(part 1 of 2)
# Autodesk Inventor assembly: ATLAS ASSEMBLY
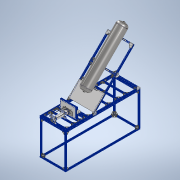
[picture p0: Inventor's stored thumbnail of the model, 180x180]
Saved by Autodesk Inventor 2021 (Build 250183000, 183)
## iProperties
Created: 2021-09-10
Part Number: ATLAS ASSEMBLY
Document SubType Name: Assembly
Designer: Alex Clay
Author: Alex Clay
## Documents named in this file (38)
- C:\Users\alexc\Embry-Riddle Aeronautical University\Kingsberry, Kyle A. - Odyssey\ATLAS V1\ATLAS ASSEMBLY.iam
- C:\Users\alexc\Embry-Riddle Aeronautical University\Kingsberry, Kyle A. - Odyssey\ATLAS V1\4040 6ft.ipt
- C:\Users\alexc\Embry-Riddle Aeronautical University\Kingsberry, Kyle A. - Odyssey\ATLAS V1\4040 3.5ft.ipt
- C:\Users\alexc\Embry-Riddle Aeronautical University\Kingsberry, Kyle A. - Odyssey\ATLAS V1\4040 2.5ft.ipt
- C:\Users\alexc\Embry-Riddle Aeronautical University\Kingsberry, Kyle A. - Odyssey\ATLAS V1\4080 6ft.ipt
- C:\Users\alexc\Embry-Riddle Aeronautical University\Kingsberry, Kyle A. - Odyssey\ATLAS V1\4 Hole Bracket.ipt
- C:\Users\alexc\Embry-Riddle Aeronautical University\Kingsberry, Kyle A. - Odyssey\ATLAS V1\4040 1ft.ipt
- C:\Users\alexc\Embry-Riddle Aeronautical University\Kingsberry, Kyle A. - Odyssey\ATLAS V1\4040 1.5ft.ipt
- C:\Users\alexc\Embry-Riddle Aeronautical University\Kingsberry, Kyle A. - Odyssey\ATLAS V1\45 Plate.ipt
- C:\Users\alexc\Embry-Riddle Aeronautical University\Kingsberry, Kyle A. - Odyssey\ATLAS V1\4040 angled.ipt
- C:\Users\alexc\Embry-Riddle Aeronautical University\Kingsberry, Kyle A. - Odyssey\ATLAS V1\4080 2.5ft.ipt
- C:\Users\alexc\Embry-Riddle Aeronautical University\Kingsberry, Kyle A. - Odyssey\ATLAS V1\90 Plate.ipt
- C:\Users\alexc\Embry-Riddle Aeronautical University\Kingsberry, Kyle A. - Odyssey\ATLAS V1\ODSY-0007-003.ipt
- C:\Users\alexc\Embry-Riddle Aeronautical University\Kingsberry, Kyle A. - Odyssey\ATLAS V1\Odyssey Bushing.ipt
- C:\Users\alexc\Embry-Riddle Aeronautical University\Kingsberry, Kyle A. - Odyssey\ATLAS V1\ODSY-0007-001.ipt
- C:\Users\alexc\Embry-Riddle Aeronautical University\Kingsberry, Kyle A. - Odyssey\ATLAS V1\8080 2.5ft.ipt
- C:\Users\alexc\Embry-Riddle Aeronautical University\Kingsberry, Kyle A. - Odyssey\ATLAS V1\ODSY-0007-002.ipt
- C:\Users\alexc\Embry-Riddle Aeronautical University\Kingsberry, Kyle A. - Odyssey\ATLAS V1\ODSY-0003 (COMBUSTION CHAMBER)\ODSY-0003.iam
- C:\Users\alexc\Embry-Riddle Aeronautical University\Kingsberry, Kyle A. - Odyssey\ATLAS V1\Load Cell.ipt
- C:\Users\alexc\Embry-Riddle Aeronautical University\Kingsberry, Kyle A. - Odyssey\ATLAS V1\ODSY-0007-004.ipt
- C:\Users\alexc\Embry-Riddle Aeronautical University\Kingsberry, Kyle A. - Odyssey\ATLAS V1\95412A566 Short Threaded Rod.ipt
- C:\Users\alexc\Embry-Riddle Aeronautical University\Kingsberry, Kyle A. - Odyssey\ATLAS V1\98804A029 Long Threaded Rod.ipt
- C:\Users\alexc\Embry-Riddle Aeronautical University\Kingsberry, Kyle A. - Odyssey\ATLAS V1\92196A801 Load Cell Bolt.ipt
- C:\Users\alexc\Embry-Riddle Aeronautical University\Kingsberry, Kyle A. - Odyssey\ATLAS V1\92141A029 0.25 Washer.ipt
- C:\Users\alexc\Embry-Riddle Aeronautical University\Kingsberry, Kyle A. - Odyssey\ATLAS V1\91292A209 Bottom Holder Screw.ipt
- C:\Users\alexc\Embry-Riddle Aeronautical University\Kingsberry, Kyle A. - Odyssey\ATLAS V1\98689A116 Bottom Holder Washer.ipt
- C:\Users\alexc\Embry-Riddle Aeronautical University\Kingsberry, Kyle A. - Odyssey\ATLAS V1\91845A029 0.25 Nut.ipt
- C:\Users\alexc\Embry-Riddle Aeronautical University\Kingsberry, Kyle A. - Odyssey\ATLAS V1\92510A475 Spacer.ipt
- C:\Users\alexc\Embry-Riddle Aeronautical University\Kingsberry, Kyle A. - Odyssey\ATLAS V1\92196A551 Engine Bolts.ipt
- C:\Users\alexc\Embry-Riddle Aeronautical University\Kingsberry, Kyle A. - Odyssey\ATLAS V1\90945A760 Washers For Engine.ipt
- C:\Users\alexc\Embry-Riddle Aeronautical University\Kingsberry, Kyle A. - Odyssey\ATLAS V1\91831A029 Lock Nuts For Engine.ipt
- C:\Users\alexc\Embry-Riddle Aeronautical University\Kingsberry, Kyle A. - Odyssey\ATLAS V1\Tank Uprights.ipt
- C:\Users\alexc\Embry-Riddle Aeronautical University\Kingsberry, Kyle A. - Odyssey\ATLAS V1\Tank Holder.ipt
- C:\Users\alexc\Embry-Riddle Aeronautical University\Kingsberry, Kyle A. - Odyssey\ATLAS V1\Tank Upright Support.ipt
- C:\Users\alexc\Embry-Riddle Aeronautical University\Kingsberry, Kyle A. - Odyssey\ATLAS V1\45 splicer.ipt
- C:\Users\alexc\Embry-Riddle Aeronautical University\Kingsberry, Kyle A. - Odyssey\ATLAS V1\40-4340.ipt
- C:\Users\alexc\Embry-Riddle Aeronautical University\Kingsberry, Kyle A. - Odyssey\ATLAS V1\Odyssey Fluids Panel.ipt
- C:\Users\alexc\Embry-Riddle Aeronautical University\Kingsberry, Kyle A. - Odyssey\ATLAS V1\ODSY-0004 (TANK)\Weld Assembly.iam
## Components (292 placed, 37 different names)
1. 4040 6ft:1 — Flush:3, Flush:4, Flush:7, Flush:8, Mate:3, Flush:11, Flush:12, Mate:5, Mate:10, Mate:28, Mate:31, Flush:39, Mate:33, Mate:36, Flush:42
2. 4040 6ft:2 — Flush:1, Mate:1, Flush:2, Flush:3, Flush:4, Flush:5, Flush:6, Mate:2, Flush:9, Flush:10, Mate:4, Mate:6, Flush:13, Flush:14, Mate:9, Flush:19, Flush:20, Mate:20, Mate:25, Mate:39, Flush:43, Mate:42
3. 4040 3.5ft:1 — Flush:7, Flush:8, Mate:3, Mate:12, Flush:23, Flush:24, Mate:27, Flush:37, Mate:29, Flush:38, Flush:49, Mate:52, Flush:93
4. 4040 3.5ft:2 — Flush:5, Flush:6, Mate:2, Flush:21, Flush:22, Mate:11, Mate:21, Flush:34, Mate:22, Flush:35, Mate:44, Flush:46, Flush:92, Flush:94
5. 4040 3.5ft:3 — Flush:9, Flush:10, Mate:4, Mate:38, Mate:40, Mate:56, Mate:59, Flush:99
6. 4040 3.5ft:4 — Flush:11, Flush:12, Mate:5, Mate:32, Flush:40, Mate:34, Mate:65, Mate:67, Flush:57, Flush:95, Flush:96
7. 4040 2.5ft:1 — Mate:6, Flush:13, Flush:14, Mate:35, Flush:41, Mate:37, Mate:41, Flush:44, Mate:43, Flush:45
8. 4040 2.5ft:2 — Mate:9, Flush:19, Flush:20, Mate:10, Mate:23, Mate:24, Flush:36, Mate:26, Mate:30
9. 4080 6ft:1 — Flush:21, Flush:22, Mate:11, Mate:15, Flush:29, Mate:17, Flush:31, Mate:45, Mate:46, Mate:48, Flush:48, Flush:52, Mate:58, Flush:53, Mate:60, Mate:70, Mate:71, Mate:82, Mate:83, Mate:84, Mate:85, Mate:86, Mate:87, Flush:98, Flush:100, Flush:101, Mate:204, Flush:102, Flush:103, Mate:207, Flush:104, Flush:105, Flush:108, Flush:109, Mate:212, Flush:112, Mate:217, Flush:113, Mate:241, Mate:242, Flush:122, Flush:123, Mate:257, Mate:259, Mate:261, Mate:263, Mate:492, Mate:518, Mate:545, Mate:584, Mate:585, Mate:586
10. 4080 6ft:2 — Mate:12, Flush:23, Flush:24, Mate:50, Mate:53, Flush:50, Mate:55, Mate:62, Mate:66, Mate:98, Mate:99, Mate:102, Mate:103, Mate:104, Mate:105, Mate:106, Mate:107, Flush:91, Flush:97, Flush:106, Flush:107, Flush:110, Flush:111, Mate:245, Mate:247, Mate:249, Mate:251, Mate:493, Mate:494, Mate:495, Mate:520, Mate:544, Mate:583, Mate:588, Mate:589, Flush:187
11. 4040 2.5ft:5 — Mate:15, Flush:29, Mate:68, Mate:69, Flush:58, Flush:59, Mate:88, Mate:89, Flush:76, Flush:77, Mate:184, Mate:185, Mate:289
12. 4040 2.5ft:6 — Mate:17, Flush:31, Mate:76, Mate:77, Flush:62, Flush:63, Mate:94, Mate:95, Flush:68, Flush:69
13. 4 Hole Bracket:1 — Mate:24, Mate:25, Flush:36
14. 4 Hole Bracket:2 — Mate:22, Mate:23, Flush:35
15. 4 Hole Bracket:3 — Mate:20, Mate:21, Flush:34
16. 4 Hole Bracket:4 — Mate:44, Mate:45, Flush:46
17. 4 Hole Bracket:5 — Mate:48, Flush:48, Mate:205
18. 4 Hole Bracket:6 — Mate:46, Flush:92, Flush:94
19. 4 Hole Bracket:7 — Mate:30, Mate:31, Flush:39
20. 4 Hole Bracket:8 — Mate:28, Mate:29, Flush:38
21. 4 Hole Bracket:9 — Mate:26, Mate:27, Flush:37
22. 4 Hole Bracket:10 — Mate:34, Mate:35, Flush:41
23. 4 Hole Bracket:11 — Mate:38, Mate:39, Flush:43
24. 4 Hole Bracket:12 — Mate:32, Mate:33, Flush:40
25. 4 Hole Bracket:13 — Mate:36, Mate:37, Flush:42
26. 4 Hole Bracket:14 — Mate:40, Mate:41, Flush:44
27. 4 Hole Bracket:15 — Mate:42, Mate:43, Flush:45
28. 4 Hole Bracket:16 — Mate:62, Flush:97, Mate:209
29. 4 Hole Bracket:17 — Mate:65, Flush:95, Flush:96
30. 4 Hole Bracket:18 — Mate:66, Mate:67, Flush:57
31. 4 Hole Bracket:19 — Mate:60, Flush:98, Mate:208
32. 4 Hole Bracket:20 — Mate:58, Mate:59, Flush:53
33. 4 Hole Bracket:21 — Mate:56, Flush:52, Flush:99
34. 4 Hole Bracket:22 — Mate:50, Flush:49, Flush:93
35. 4 Hole Bracket:23 — Mate:55, Flush:91, Mate:206
36. 4 Hole Bracket:24 — Mate:52, Mate:53, Flush:50
37. 4 Hole Bracket:25 — Mate:88, Mate:107, Flush:76
38. 4 Hole Bracket:26 — Mate:89, Mate:106, Flush:77
39. 4 Hole Bracket:27 — Mate:105, Flush:111, Mate:220
40. 4 Hole Bracket:28 — Mate:104, Flush:110, Mate:221
41. 4 Hole Bracket:29 — Mate:103, Flush:107, Mate:215
42. 4 Hole Bracket:30 — Mate:102, Flush:106, Mate:216
43. 4 Hole Bracket:31 — Mate:94, Mate:99, Flush:69
44. 4 Hole Bracket:32 — Mate:95, Mate:98, Flush:68
45. 4 Hole Bracket:37 — Mate:77, Mate:83, Flush:63
46. 4 Hole Bracket:38 — Mate:76, Mate:82, Flush:62
47. 4 Hole Bracket:39 — Mate:85, Flush:105, Mate:214
48. 4 Hole Bracket:40 — Mate:84, Flush:104, Mate:213
49. 4 Hole Bracket:41 — Mate:87, Flush:109, Mate:219
50. 4 Hole Bracket:42 — Mate:86, Flush:108, Mate:218
51. 4 Hole Bracket:43 — Mate:69, Mate:71, Flush:58
52. 4 Hole Bracket:44 — Mate:68, Mate:70, Flush:59
53. 4040 1ft:1 — Mate:110, Flush:80, Flush:81, Mate:133, Flush:85, Mate:167, Mate:176, Mate:177, Mate:178, Mate:210, Mate:229
54. 4040 1ft:2 — Mate:111, Flush:82, Flush:83, Mate:112, Mate:113, Mate:129, Mate:173, Mate:211, Mate:227, Flush:116, Mate:228, Flush:119, Mate:232
55. 4040 1.5ft:1 — Mate:110, Flush:80, Flush:81, Mate:111, Flush:82, Flush:83, Mate:186, Mate:187, Flush:117, Flush:118
56. 45 Plate:2 — Mate:112, Mate:113, Mate:126, Mate:127, Mate:128
57. 4040 angled:1 — Mate:126, Mate:127, Mate:128, Mate:129, Mate:226, Mate:343
58. 4040 angled:2 — Mate:133, Flush:85, Mate:179, Mate:533
59. 90 Plate:2 — Mate:167, Mate:210, Mate:229, Mate:230
60. 90 Plate:4 — Mate:173, Mate:211, Mate:228, Mate:231
61. 45 Plate:3 — Mate:176, Mate:177, Mate:178, Mate:179
62. ODSY-0007-003:1 — Mate:186, Mate:233, Mate:282, Mate:283, Mate:284, Mate:285, Mate:286, Mate:287, Mate:288, Angle:1, Mate:293, Mate:294, Mate:307, Mate:308, Mate:312, Mate:313, Mate:377, Mate:378, Mate:384, Mate:387, Mate:456
63. ODSY-0007-003:2 — Mate:184, Mate:185, Mate:187, Mate:195, Mate:196, Mate:197, Mate:279, Mate:280, Mate:281, Mate:289, Mate:291, Mate:292, Mate:309, Mate:310, Mate:311, Mate:314, Mate:376, Mate:379, Mate:385, Mate:386, Mate:456
64. Odyssey Bushing:1 — Mate:195, Mate:196, Mate:197
65. 8080 2.5ft:1 — Flush:100, Flush:101, Mate:204, Mate:205, Mate:206, Mate:233, Mate:288
66. 8080 2.5ft:2 — Flush:102, Flush:103, Mate:207, Mate:208, Mate:209
67. 8080 2.5ft:3 — Mate:217, Flush:113, Mate:218, Mate:219, Mate:220, Mate:221, Mate:226, Mate:343, Mate:533
68. 4080 2.5ft:1 — Mate:212, Flush:112, Mate:213, Mate:214, Mate:215, Mate:216, Mate:227, Flush:116, Mate:230, Mate:231, Flush:117
69. ODSY-0007-001:1 — Flush:118, Flush:119, Mate:232, Mate:275, Mate:276, Mate:331, Mate:332, Mate:334, Mate:337, Mate:368, Mate:369, Mate:370, Mate:371, Mate:466, Mate:472
70. ODSY-0007-002:1 — Mate:268, Mate:269, Mate:342, Mate:467, Mate:468, Mate:469, Mate:470, Mate:481, Mate:484, Mate:486
71. 4040 2.5ft:8 — Mate:241, Flush:123, Mate:244, Flush:124, Mate:246, Flush:125, Mate:256, Flush:130, Mate:258, Flush:131
72. 4040 2.5ft:9 — Mate:242, Flush:122, Mate:248, Flush:126, Mate:250, Flush:127, Mate:260, Flush:132, Mate:262, Flush:133
73. 4 Hole Bracket:45 — Mate:244, Flush:124, Mate:245
74. 4 Hole Bracket:46 — Mate:246, Flush:125, Mate:247
75. 4 Hole Bracket:48 — Mate:248, Flush:126, Mate:249
76. 4 Hole Bracket:49 — Mate:250, Flush:127, Mate:251
77. 4 Hole Bracket:51 — Mate:258, Flush:131, Mate:259
78. 4 Hole Bracket:52 — Mate:256, Flush:130, Mate:257
79. 4 Hole Bracket:55 — Mate:262, Flush:133, Mate:263
80. 4 Hole Bracket:56 — Mate:260, Flush:132, Mate:261
81. Combustion Chamber Assembly:1 [sub-assembly] — Mate:268, Mate:269, Mate:488, Mate:489
82. Load Cell:1 — Mate:275, Mate:276, Mate:469
83. Odyssey Bushing:2 — Mate:279, Mate:280, Mate:281
84. Odyssey Bushing:3 — Mate:285, Mate:286, Mate:287
85. Odyssey Bushing:4 — Mate:282, Mate:283, Mate:284
86. ODSY-0007-004:1 — Angle:1, Mate:293, Mate:294, Mate:295, Mate:296, Mate:297, Mate:298, Mate:299, Mate:300, Mate:350, Mate:351, Mate:357, Mate:359, Mate:374, Mate:375, Mate:471, Mate:476, Mate:478
87. ODSY-0007-004:2 — Mate:291, Mate:292, Mate:301, Mate:302, Mate:303, Mate:304, Mate:305, Mate:306, Mate:319, Mate:320, Mate:345, Mate:347, Mate:353, Mate:355, Mate:372, Mate:373, Mate:474, Mate:480
88. Odyssey Bushing:5 — Mate:298, Mate:299, Mate:300
89. Odyssey Bushing:6 — Mate:295, Mate:296, Mate:297
90. Odyssey Bushing:7 — Mate:304, Mate:305, Mate:306
91. Odyssey Bushing:8 — Mate:301, Mate:302, Mate:303
92. 95412A566 Short Threaded Rod:1 — Mate:310, Mate:311, Mate:344, Mate:400, Mate:401, Mate:473
93. 95412A566 Short Threaded Rod:2 — Mate:307, Mate:312, Mate:348, Mate:392, Mate:393, Mate:475
94. 95412A566 Short Threaded Rod:3 — Mate:309, Mate:314, Mate:346, Mate:404, Mate:405, Mate:479
95. 95412A566 Short Threaded Rod:4 — Mate:308, Mate:313, Mate:349, Mate:397, Mate:398, Mate:477
96. 98804A029 Long Threaded Rod:1 — Mate:319, Mate:352, Mate:354, Mate:356, Mate:358, Mate:366, Mate:367, Mate:408, Mate:409, Mate:414, Mate:415, Mate:424, Mate:425, Mate:426, Mate:427, Mate:444, Mate:445, Mate:446, Mate:447, Flush:150, Flush:151, Flush:152, Mate:471, Mate:472
97. 98804A029 Long Threaded Rod:2 — Mate:320, Mate:360, Mate:361, Mate:362, Mate:363, Mate:364, Mate:365, Mate:410, Mate:411, Mate:412, Mate:413, Mate:428, Mate:429, Mate:430, Mate:431, Mate:440, Mate:441, Mate:442, Mate:443, Flush:150
98. 92196A801 Load Cell Bolt:1 — Mate:331, Mate:333, Mate:335, Mate:341, Mate:457, Mate:458, Mate:465, Mate:467
99. 92196A801 Load Cell Bolt:2 — Mate:332, Mate:336, Mate:338, Mate:339, Mate:461, Mate:463, Mate:468
100. 92141A029 0.25 Washer:1 — Mate:333, Mate:334, Mate:335
101. 92141A029 0.25 Washer:2 — Mate:336, Mate:337, Mate:338
102. 92141A029 0.25 Washer:3 — Mate:341, Mate:342, Mate:459
103. 92141A029 0.25 Washer:4 — Mate:339, Mate:462, Mate:470
104. 92141A029 0.25 Washer:5 — Mate:346, Mate:347, Mate:407
105. 92141A029 0.25 Washer:6 — Mate:348, Mate:351, Mate:394
106. 92141A029 0.25 Washer:7 — Mate:344, Mate:345, Mate:403
107. 92141A029 0.25 Washer:8 — Mate:349, Mate:350, Mate:396
108. 92141A029 0.25 Washer:9 — Mate:356, Mate:357, Mate:418
109. 92141A029 0.25 Washer:10 — Mate:358, Mate:359, Mate:416
110. 92141A029 0.25 Washer:11 — Mate:354, Mate:355, Mate:434
111. 92141A029 0.25 Washer:12 — Mate:352, Mate:353, Mate:432
112. 92141A029 0.25 Washer:13 — Mate:360, Mate:374, Mate:420
113. 92141A029 0.25 Washer:14 — Mate:361, Mate:375, Mate:422
114. 92141A029 0.25 Washer:15 — Mate:362, Mate:372, Mate:436
115. 92141A029 0.25 Washer:16 — Mate:363, Mate:373, Mate:438
116. 92141A029 0.25 Washer:17 — Mate:364, Mate:368, Mate:455
117. 92141A029 0.25 Washer:18 — Mate:365, Mate:371, Mate:451
118. 92141A029 0.25 Washer:19 — Mate:367, Mate:369, Mate:452
119. 92141A029 0.25 Washer:20 — Mate:366, Mate:370, Mate:449
120. 91292A209 Bottom Holder Screw:1 — Mate:377, Mate:381, Mate:388
121. 91292A209 Bottom Holder Screw:2 — Mate:376, Mate:380, Mate:389
122. 91292A209 Bottom Holder Screw:3 — Mate:379, Mate:383, Mate:391
123. 91292A209 Bottom Holder Screw:4 — Mate:378, Mate:382, Mate:390
124. 98689A116 Bottom Holder Washer:1 — Mate:381, Mate:387, Mate:388
125. 98689A116 Bottom Holder Washer:2 — Mate:380, Mate:386, Mate:389
126. 98689A116 Bottom Holder Washer:3 — Mate:382, Mate:384, Mate:390
127. 98689A116 Bottom Holder Washer:4 — Mate:383, Mate:385, Mate:391
128. 91845A029 0.25 Nut:1 — Mate:404, Mate:406
129. 91845A029 0.25 Nut:2 — Mate:393, Flush:136, Mate:395
130. 91845A029 0.25 Nut:3 — Mate:400, Flush:138, Mate:402, Mate:403
131. 91845A029 0.25 Nut:4 — Mate:392, Flush:136, Mate:394, Mate:395
132. 91845A029 0.25 Nut:5 — Mate:398, Flush:137, Mate:399
133. 91845A029 0.25 Nut:6 — Mate:405, Mate:406, Mate:407
134. 91845A029 0.25 Nut:7 — Mate:401, Flush:138, Mate:402
135. 91845A029 0.25 Nut:8 — Mate:396, Mate:397, Flush:137, Mate:399
136. 91845A029 0.25 Nut:9 — Mate:415, Flush:139, Mate:416, Mate:417
137. 91845A029 0.25 Nut:10 — Mate:414, Flush:139, Mate:417
138. 91845A029 0.25 Nut:11 — Mate:413, Mate:421, Flush:141
139. 91845A029 0.25 Nut:12 — Mate:412, Mate:420, Mate:421, Flush:141
140. 91845A029 0.25 Nut:13 — Mate:410, Mate:422, Mate:423, Flush:142
141. 91845A029 0.25 Nut:14 — Mate:411, Mate:423, Flush:142
142. 91845A029 0.25 Nut:15 — Mate:408, Mate:418, Mate:419, Flush:140
143. 91845A029 0.25 Nut:16 — Mate:409, Mate:419, Flush:140, Flush:151
144. 91845A029 0.25 Nut:17 — Mate:424, Flush:146, Mate:432, Mate:433
145. 91845A029 0.25 Nut:18 — Mate:425, Flush:146, Mate:433
146. 91845A029 0.25 Nut:19 — Mate:426, Flush:145, Mate:434, Mate:435
147. 91845A029 0.25 Nut:20 — Mate:427, Flush:145, Mate:435
148. 91845A029 0.25 Nut:21 — Mate:429, Flush:144, Mate:437
149. 91845A029 0.25 Nut:22 — Mate:428, Flush:144, Mate:436, Mate:437
150. 91845A029 0.25 Nut:23 — Mate:431, Flush:143, Mate:438, Mate:439
151. 91845A029 0.25 Nut:24 — Mate:430, Flush:143, Mate:439
152. 91845A029 0.25 Nut:25 — Mate:445, Mate:453
153. 91845A029 0.25 Nut:26 — Mate:444, Mate:452, Mate:453
154. 91845A029 0.25 Nut:27 — Mate:447, Flush:147, Mate:448, Mate:449
155. 91845A029 0.25 Nut:28 — Mate:446, Flush:147, Mate:448, Flush:152
156. 91845A029 0.25 Nut:29 — Mate:440, Mate:450, Flush:148, Mate:451
157. 91845A029 0.25 Nut:30 — Mate:441, Mate:450, Flush:148
158. 91845A029 0.25 Nut:31 — Mate:442, Mate:454, Flush:149, Mate:455
159. 91845A029 0.25 Nut:32 — Mate:443, Mate:454, Flush:149
160. 91845A029 0.25 Nut:33 — Mate:461, Mate:462, Flush:154, Mate:464
161. 91845A029 0.25 Nut:34 — Mate:463, Flush:154, Mate:464
162. 91845A029 0.25 Nut:35 — Mate:457, Flush:153, Mate:459, Mate:460
163. 91845A029 0.25 Nut:36 — Mate:458, Flush:153, Mate:460
164. Load Cell:2 — Mate:465, Mate:466
165. 92510A475 Spacer:1 — Mate:475, Mate:476
166. 92510A475 Spacer:2 — Mate:473, Mate:474
167. 92510A475 Spacer:3 — Mate:479, Mate:480
168. 92510A475 Spacer:4 — Mate:477, Mate:478
169. 45 Plate:4 — Mate:493, Flush:155, Flush:156, Mate:494, Mate:495, Mate:496, Mate:498, Mate:499
170. 45 Plate:5 — Mate:492, Flush:155, Flush:156, Mate:497, Mate:501, Mate:502, Mate:503
171. Tank Uprights:1 — Mate:496, Mate:498, Mate:499, Mate:506, Flush:159, Flush:161, Flush:163, Mate:515, Mate:536, Mate:537, Mate:542, Flush:169, Flush:170, Mate:552, Flush:176, Mate:556, Mate:561, Flush:180, Mate:563, Flush:181, Mate:567, Flush:183, Mate:570, Mate:571, Mate:572, Mate:573, Mate:578, Flush:185
172. Tank Uprights:2 — Mate:497, Mate:501, Mate:502, Mate:503, Mate:507, Flush:160, Flush:164, Mate:516, Mate:528, Mate:539, Mate:540, Mate:543, Flush:171, Flush:172, Mate:546, Flush:173, Mate:551, Mate:554, Flush:177, Mate:559, Flush:179, Mate:565, Flush:182, Mate:569, Flush:184, Mate:577
173. 4040 2.5ft:12 — Mate:507, Flush:160, Mate:508, Mate:512, Flush:161, Mate:532, Mate:550, Flush:175, Mate:553, Mate:574, Mate:575, Mate:576
174. 4040 2.5ft:13 — Mate:506, Flush:159, Mate:509, Mate:513, Mate:532, Mate:555, Mate:557, Flush:178, Mate:558, Mate:560
175. Tank Holder:1 — Mate:509, Mate:513, Mate:528, Mate:580, Mate:581
176. Tank Holder:2 — Mate:508, Mate:512, Mate:580, Mate:582
177. Tank Upright Support:1 — Flush:164, Mate:516, Mate:517, Flush:165, Flush:166, Mate:535, Mate:541, Mate:587
178. Tank Upright Support:2 — Flush:163, Mate:515, Mate:519, Flush:167, Flush:168, Mate:534, Mate:538, Mate:590
179. 45 splicer:1 — Mate:517, Flush:165, Flush:166, Mate:518
180. 45 splicer:2 — Mate:519, Flush:167, Flush:168, Mate:520
181. 40-4340:1 — Mate:534, Mate:536, Mate:537, Mate:538
182. 40-4340:2 — Mate:535, Mate:539, Mate:540, Mate:541
183. 45 splicer:3 — Mate:543, Flush:171, Flush:172, Mate:545
184. 45 splicer:4 — Mate:542, Flush:169, Flush:170, Mate:544, Mate:579
185. 4040 2.5ft:14 — Mate:546, Flush:173, Mate:548, Flush:174, Mate:562, Mate:564, Mate:566, Mate:568, Flush:186
186. Tank Holder:3 — Mate:548, Flush:174, Mate:581
187. 4 Hole Bracket:57 — Mate:550, Mate:551, Flush:175
188. 4 Hole Bracket:58 — Mate:552, Mate:553, Flush:176
189. 4 Hole Bracket:59 — Mate:554, Mate:555, Flush:177
190. 4 Hole Bracket:60 — Mate:568, Mate:569, Flush:184
191. 4 Hole Bracket:61 — Mate:556, Mate:557, Flush:178
192. 4 Hole Bracket:62 — Mate:560, Mate:561, Flush:180
193. 4 Hole Bracket:63 — Mate:558, Mate:559, Flush:179
194. 4 Hole Bracket:64 — Mate:562, Mate:563, Flush:181
195. 4 Hole Bracket:65 — Mate:564, Mate:565, Flush:182
196. 4 Hole Bracket:66 — Mate:566, Mate:567, Flush:183
197. 45 Plate:6 — Mate:570, Mate:571, Mate:572, Mate:573
198. 45 Plate:7 — Mate:574, Mate:575, Mate:576, Mate:577
199. Odyssey Fluids Panel:1 — Mate:578, Mate:579, Flush:185, Flush:186
200. Weld Assembly:1 [sub-assembly] — Mate:582
201. 45 Plate:8 — Mate:584, Mate:585, Mate:586, Mate:587
202. 45 Plate:9 — Mate:583, Mate:588, Mate:589, Mate:590, Flush:187
203. 92196A551 Engine Bolts:1 — Mate:481, Mate:482, Mate:483, Mate:485, Mate:487, Mate:490
204. 90945A760 Washers For Engine:1 — Mate:482, Mate:483, Mate:484
205. 90945A760 Washers For Engine:2 — Mate:485, Mate:486, Mate:488
206. 90945A760 Washers For Engine:3 — Mate:487, Mate:489, Mate:491
207. 91831A029 Lock Nuts For Engine:1 — Mate:490, Mate:491
208. 92196A551 Engine Bolts:2
209. 90945A760 Washers For Engine:4
210. 90945A760 Washers For Engine:5
211. 90945A760 Washers For Engine:6
212. 91831A029 Lock Nuts For Engine:2
213. 92196A551 Engine Bolts:3
214. 90945A760 Washers For Engine:7
215. 90945A760 Washers For Engine:8
216. 90945A760 Washers For Engine:9
217. 91831A029 Lock Nuts For Engine:3
218. 92196A551 Engine Bolts:4
219. 90945A760 Washers For Engine:10
220. 90945A760 Washers For Engine:11
221. 90945A760 Washers For Engine:12
222. 91831A029 Lock Nuts For Engine:4
223. 92196A551 Engine Bolts:5
224. 90945A760 Washers For Engine:13
225. 90945A760 Washers For Engine:14
226. 90945A760 Washers For Engine:15
227. 91831A029 Lock Nuts For Engine:5
228. 92196A551 Engine Bolts:6
229. 90945A760 Washers For Engine:16
230. 90945A760 Washers For Engine:17
231. 90945A760 Washers For Engine:18
232. 91831A029 Lock Nuts For Engine:6
233. 92196A551 Engine Bolts:7
234. 90945A760 Washers For Engine:19
235. 90945A760 Washers For Engine:20
236. 90945A760 Washers For Engine:21
237. 91831A029 Lock Nuts For Engine:7
238. 92196A551 Engine Bolts:8
239. 90945A760 Washers For Engine:22
240. 90945A760 Washers For Engine:23
241. 90945A760 Washers For Engine:24
242. 91831A029 Lock Nuts For Engine:8
243. 92196A551 Engine Bolts:9
244. 90945A760 Washers For Engine:25
245. 90945A760 Washers For Engine:26
246. 90945A760 Washers For Engine:27
247. 91831A029 Lock Nuts For Engine:9
248. 92196A551 Engine Bolts:10
249. 90945A760 Washers For Engine:28
250. 90945A760 Washers For Engine:29
251. 90945A760 Washers For Engine:30
252. 91831A029 Lock Nuts For Engine:10
253. 92196A551 Engine Bolts:11
254. 90945A760 Washers For Engine:31
255. 90945A760 Washers For Engine:32
256. 90945A760 Washers For Engine:33
257. 91831A029 Lock Nuts For Engine:11
258. 92196A551 Engine Bolts:12
259. 90945A760 Washers For Engine:34
260. 90945A760 Washers For Engine:35
261. 90945A760 Washers For Engine:36
262. 91831A029 Lock Nuts For Engine:12
263. 92196A551 Engine Bolts:13
264. 90945A760 Washers For Engine:37
265. 90945A760 Washers For Engine:38
266. 90945A760 Washers For Engine:39
267. 91831A029 Lock Nuts For Engine:13
268. 92196A551 Engine Bolts:14
269. 90945A760 Washers For Engine:40
270. 90945A760 Washers For Engine:41
271. 90945A760 Washers For Engine:42
272. 91831A029 Lock Nuts For Engine:14
273. 92196A551 Engine Bolts:15
274. 90945A760 Washers For Engine:43
275. 90945A760 Washers For Engine:44
276. 90945A760 Washers For Engine:45
277. 91831A029 Lock Nuts For Engine:15
278. 92196A551 Engine Bolts:16
279. 90945A760 Washers For Engine:46
280. 90945A760 Washers For Engine:47
281. 90945A760 Washers For Engine:48
282. 91831A029 Lock Nuts For Engine:16
283. 92196A551 Engine Bolts:17
284. 90945A760 Washers For Engine:49
285. 90945A760 Washers For Engine:50
286. 90945A760 Washers For Engine:51
287. 91831A029 Lock Nuts For Engine:17
288. 92196A551 Engine Bolts:18
289. 90945A760 Washers For Engine:52
290. 90945A760 Washers For Engine:53
291. 90945A760 Washers For Engine:54
292. 91831A029 Lock Nuts For Engine:18
## Component patterns: (18 elements, first: 92196A551 Engine Bolts:1 + 90945A760 Washers For Engine:1 + 90945A760 Washers For Engine:2 + 90945A760 Washers For Engine:3 + 91831A029 Lock Nuts For Engine:1)
## Relationships (565: Mate 424, Flush 140, Angle 1)
- Flush:1: 4040 6ft:2
- Mate:1: 4040 6ft:2
- Flush:2: 4040 6ft:2
- Flush:3: 4040 6ft:1 ↔ 4040 6ft:2
- Flush:4: 4040 6ft:1 ↔ 4040 6ft:2
- Flush:5: 4040 6ft:2 ↔ 4040 3.5ft:2
- Flush:6: 4040 6ft:2 ↔ 4040 3.5ft:2
- Mate:2: 4040 6ft:2 ↔ 4040 3.5ft:2
- Flush:7: 4040 6ft:1 ↔ 4040 3.5ft:1
- Flush:8: 4040 6ft:1 ↔ 4040 3.5ft:1
- Mate:3: 4040 6ft:1 ↔ 4040 3.5ft:1
- Flush:9: 4040 6ft:2 ↔ 4040 3.5ft:3
- Flush:10: 4040 6ft:2 ↔ 4040 3.5ft:3
- Mate:4: 4040 6ft:2 ↔ 4040 3.5ft:3
- Flush:11: 4040 6ft:1 ↔ 4040 3.5ft:4
- Flush:12: 4040 6ft:1 ↔ 4040 3.5ft:4
- Mate:5: 4040 6ft:1 ↔ 4040 3.5ft:4
- Mate:6: 4040 6ft:2 ↔ 4040 2.5ft:1
- Flush:13: 4040 6ft:2 ↔ 4040 2.5ft:1
- Flush:14: 4040 6ft:2 ↔ 4040 2.5ft:1
- Mate:9: 4040 6ft:2 ↔ 4040 2.5ft:2
- Flush:19: 4040 6ft:2 ↔ 4040 2.5ft:2
- Flush:20: 4040 6ft:2 ↔ 4040 2.5ft:2
- Mate:10: 4040 6ft:1 ↔ 4040 2.5ft:2
- Flush:21: 4040 3.5ft:2 ↔ 4080 6ft:1
- Flush:22: 4040 3.5ft:2 ↔ 4080 6ft:1
- Mate:11: 4040 3.5ft:2 ↔ 4080 6ft:1
- Mate:12: 4040 3.5ft:1 ↔ 4080 6ft:2
- Flush:23: 4040 3.5ft:1 ↔ 4080 6ft:2
- Flush:24: 4040 3.5ft:1 ↔ 4080 6ft:2
- Mate:15: 4080 6ft:1 ↔ 4040 2.5ft:5
- Flush:29: 4080 6ft:1 ↔ 4040 2.5ft:5
- Mate:17: 4080 6ft:1 ↔ 4040 2.5ft:6
- Flush:31: 4080 6ft:1 ↔ 4040 2.5ft:6
- Mate:20: 4040 6ft:2 ↔ 4 Hole Bracket:3
- Mate:21: 4040 3.5ft:2 ↔ 4 Hole Bracket:3
- Flush:34 (-2 mm): 4040 3.5ft:2 ↔ 4 Hole Bracket:3
- Mate:22: 4040 3.5ft:2 ↔ 4 Hole Bracket:2
- Mate:23: 4040 2.5ft:2 ↔ 4 Hole Bracket:2
- Flush:35 (2 mm): 4040 3.5ft:2 ↔ 4 Hole Bracket:2
- Mate:24: 4040 2.5ft:2 ↔ 4 Hole Bracket:1
- Mate:25: 4040 6ft:2 ↔ 4 Hole Bracket:1
- Flush:36 (2 mm): 4040 2.5ft:2 ↔ 4 Hole Bracket:1
- Mate:26: 4040 2.5ft:2 ↔ 4 Hole Bracket:9
- Mate:27: 4040 3.5ft:1 ↔ 4 Hole Bracket:9
- Flush:37 (-2 mm): 4040 3.5ft:1 ↔ 4 Hole Bracket:9
- Mate:28: 4040 6ft:1 ↔ 4 Hole Bracket:8
- Mate:29: 4040 3.5ft:1 ↔ 4 Hole Bracket:8
- Flush:38 (2 mm): 4040 3.5ft:1 ↔ 4 Hole Bracket:8
- Mate:30: 4040 2.5ft:2 ↔ 4 Hole Bracket:7
- Mate:31: 4040 6ft:1 ↔ 4 Hole Bracket:7
- Flush:39 (2 mm): 4040 6ft:1 ↔ 4 Hole Bracket:7
- Mate:32: 4040 3.5ft:4 ↔ 4 Hole Bracket:12
- Mate:33: 4040 6ft:1 ↔ 4 Hole Bracket:12
- Flush:40 (-2 mm): 4040 3.5ft:4 ↔ 4 Hole Bracket:12
- Mate:34: 4040 3.5ft:4 ↔ 4 Hole Bracket:10
- Mate:35: 4040 2.5ft:1 ↔ 4 Hole Bracket:10
- Flush:41 (2 mm): 4040 2.5ft:1 ↔ 4 Hole Bracket:10
- Mate:36: 4040 6ft:1 ↔ 4 Hole Bracket:13
- Mate:37: 4040 2.5ft:1 ↔ 4 Hole Bracket:13
- Flush:42 (2 mm): 4040 6ft:1 ↔ 4 Hole Bracket:13
- Mate:38: 4040 3.5ft:3 ↔ 4 Hole Bracket:11
- Mate:39: 4040 6ft:2 ↔ 4 Hole Bracket:11
- Flush:43 (2 mm): 4040 6ft:2 ↔ 4 Hole Bracket:11
- Mate:40: 4040 3.5ft:3 ↔ 4 Hole Bracket:14
- Mate:41: 4040 2.5ft:1 ↔ 4 Hole Bracket:14
- Flush:44 (2 mm): 4040 2.5ft:1 ↔ 4 Hole Bracket:14
- Mate:42: 4040 6ft:2 ↔ 4 Hole Bracket:15
- Mate:43: 4040 2.5ft:1 ↔ 4 Hole Bracket:15
- Flush:45 (-2 mm): 4040 2.5ft:1 ↔ 4 Hole Bracket:15
- Mate:44: 4040 3.5ft:2 ↔ 4 Hole Bracket:4
- Mate:45: 4080 6ft:1 ↔ 4 Hole Bracket:4
- Flush:46 (2 mm): 4040 3.5ft:2 ↔ 4 Hole Bracket:4
- Mate:46: 4080 6ft:1 ↔ 4 Hole Bracket:6
- Mate:48: 4080 6ft:1 ↔ 4 Hole Bracket:5
- Flush:48 (-2 mm): 4080 6ft:1 ↔ 4 Hole Bracket:5
- Mate:50: 4080 6ft:2 ↔ 4 Hole Bracket:22
- Flush:49 (2 mm): 4040 3.5ft:1 ↔ 4 Hole Bracket:22
- Mate:52: 4040 3.5ft:1 ↔ 4 Hole Bracket:24
- Mate:53: 4080 6ft:2 ↔ 4 Hole Bracket:24
- Flush:50 (2 mm): 4080 6ft:2 ↔ 4 Hole Bracket:24
- Mate:55: 4080 6ft:2 ↔ 4 Hole Bracket:23
- Mate:56: 4040 3.5ft:3 ↔ 4 Hole Bracket:21
- Flush:52 (2 mm): 4080 6ft:1 ↔ 4 Hole Bracket:21
- Mate:58: 4080 6ft:1 ↔ 4 Hole Bracket:20
- Mate:59: 4040 3.5ft:3 ↔ 4 Hole Bracket:20
- Flush:53 (2 mm): 4080 6ft:1 ↔ 4 Hole Bracket:20
- Mate:60: 4080 6ft:1 ↔ 4 Hole Bracket:19
- Mate:62: 4080 6ft:2 ↔ 4 Hole Bracket:16
- Mate:65: 4040 3.5ft:4 ↔ 4 Hole Bracket:17
- Mate:66: 4080 6ft:2 ↔ 4 Hole Bracket:18
- Mate:67: 4040 3.5ft:4 ↔ 4 Hole Bracket:18
- Flush:57 (2 mm): 4040 3.5ft:4 ↔ 4 Hole Bracket:18
- Mate:68: 4040 2.5ft:5 ↔ 4 Hole Bracket:44
- Mate:69: 4040 2.5ft:5 ↔ 4 Hole Bracket:43
- Mate:70: 4080 6ft:1 ↔ 4 Hole Bracket:44
- Mate:71: 4080 6ft:1 ↔ 4 Hole Bracket:43
- Flush:58 (2 mm): 4040 2.5ft:5 ↔ 4 Hole Bracket:43
- Flush:59 (2 mm): 4040 2.5ft:5 ↔ 4 Hole Bracket:44
- Mate:76: 4040 2.5ft:6 ↔ 4 Hole Bracket:38
- Mate:77: 4040 2.5ft:6 ↔ 4 Hole Bracket:37
- Mate:82: 4080 6ft:1 ↔ 4 Hole Bracket:38
- Flush:62 (2 mm): 4040 2.5ft:6 ↔ 4 Hole Bracket:38
- Mate:83: 4080 6ft:1 ↔ 4 Hole Bracket:37
- Flush:63 (2 mm): 4040 2.5ft:6 ↔ 4 Hole Bracket:37
- Mate:84: 4080 6ft:1 ↔ 4 Hole Bracket:40
- Mate:85: 4080 6ft:1 ↔ 4 Hole Bracket:39
- Mate:86: 4080 6ft:1 ↔ 4 Hole Bracket:42
- Mate:87: 4080 6ft:1 ↔ 4 Hole Bracket:41
- Mate:88: 4040 2.5ft:5 ↔ 4 Hole Bracket:25
- Mate:89: 4040 2.5ft:5 ↔ 4 Hole Bracket:26
- Mate:94: 4040 2.5ft:6 ↔ 4 Hole Bracket:31
- Mate:95: 4040 2.5ft:6 ↔ 4 Hole Bracket:32
- Mate:98: 4080 6ft:2 ↔ 4 Hole Bracket:32
- Flush:68 (2 mm): 4040 2.5ft:6 ↔ 4 Hole Bracket:32
- Mate:99: 4080 6ft:2 ↔ 4 Hole Bracket:31
- Flush:69 (2 mm): 4040 2.5ft:6 ↔ 4 Hole Bracket:31
- Mate:102: 4080 6ft:2 ↔ 4 Hole Bracket:30
- Mate:103: 4080 6ft:2 ↔ 4 Hole Bracket:29
- Mate:104: 4080 6ft:2 ↔ 4 Hole Bracket:28
- Mate:105: 4080 6ft:2 ↔ 4 Hole Bracket:27
- Mate:106: 4080 6ft:2 ↔ 4 Hole Bracket:26
- Mate:107: 4080 6ft:2 ↔ 4 Hole Bracket:25
- Flush:76 (2 mm): 4040 2.5ft:5 ↔ 4 Hole Bracket:25
- Flush:77 (2 mm): 4040 2.5ft:5 ↔ 4 Hole Bracket:26
- Mate:110: 4040 1ft:1 ↔ 4040 1.5ft:1
- Flush:80: 4040 1ft:1 ↔ 4040 1.5ft:1
- Flush:81: 4040 1ft:1 ↔ 4040 1.5ft:1
- Mate:111: 4040 1ft:2 ↔ 4040 1.5ft:1
- Flush:82: 4040 1ft:2 ↔ 4040 1.5ft:1
- Flush:83: 4040 1ft:2 ↔ 4040 1.5ft:1
- Mate:112: 4040 1ft:2 ↔ 45 Plate:2
- Mate:113: 4040 1ft:2 ↔ 45 Plate:2
- Mate:126: 45 Plate:2 ↔ 4040 angled:1
- Mate:127: 45 Plate:2 ↔ 4040 angled:1
- Mate:128: 45 Plate:2 ↔ 4040 angled:1
- Mate:129: 4040 1ft:2 ↔ 4040 angled:1
- Mate:133: 4040 1ft:1 ↔ 4040 angled:2
- Flush:85: 4040 1ft:1 ↔ 4040 angled:2
- Mate:167: 4040 1ft:1 ↔ 90 Plate:2
- Mate:173: 4040 1ft:2 ↔ 90 Plate:4
- Mate:176: 4040 1ft:1 ↔ 45 Plate:3
- Mate:177: 4040 1ft:1 ↔ 45 Plate:3
- Mate:178: 4040 1ft:1 ↔ 45 Plate:3
- Mate:179: 4040 angled:2 ↔ 45 Plate:3
- Mate:184: 4040 2.5ft:5 ↔ ODSY-0007-003:2
- Mate:185: 4040 2.5ft:5 ↔ ODSY-0007-003:2
- Mate:186: 4040 1.5ft:1 ↔ ODSY-0007-003:1
- Mate:187: 4040 1.5ft:1 ↔ ODSY-0007-003:2
- Mate:195: ODSY-0007-003:2 ↔ Odyssey Bushing:1
- Mate:196: ODSY-0007-003:2 ↔ Odyssey Bushing:1
- Mate:197: ODSY-0007-003:2 ↔ Odyssey Bushing:1
- Flush:91 (-2 mm): 4080 6ft:2 ↔ 4 Hole Bracket:23
- Flush:92 (2 mm): 4040 3.5ft:2 ↔ 4 Hole Bracket:6
- Flush:93: 4040 3.5ft:1 ↔ 4 Hole Bracket:22
- Flush:94: 4040 3.5ft:2 ↔ 4 Hole Bracket:6
- Flush:95 (2 mm): 4040 3.5ft:4 ↔ 4 Hole Bracket:17
- Flush:96: 4040 3.5ft:4 ↔ 4 Hole Bracket:17
- Flush:97 (2 mm): 4080 6ft:2 ↔ 4 Hole Bracket:16
- Flush:98 (2 mm): 4080 6ft:1 ↔ 4 Hole Bracket:19
- Flush:99: 4040 3.5ft:3 ↔ 4 Hole Bracket:21
- Flush:100: 4080 6ft:1 ↔ 8080 2.5ft:1
- Flush:101: 4080 6ft:1 ↔ 8080 2.5ft:1
- Mate:204: 4080 6ft:1 ↔ 8080 2.5ft:1
- Mate:205: 4 Hole Bracket:5 ↔ 8080 2.5ft:1
- Mate:206: 4 Hole Bracket:23 ↔ 8080 2.5ft:1
- Flush:102: 4080 6ft:1 ↔ 8080 2.5ft:2
- Flush:103: 4080 6ft:1 ↔ 8080 2.5ft:2
- Mate:207: 4080 6ft:1 ↔ 8080 2.5ft:2
- Mate:208: 4 Hole Bracket:19 ↔ 8080 2.5ft:2
- Mate:209: 4 Hole Bracket:16 ↔ 8080 2.5ft:2
- Mate:210: 4040 1ft:1 ↔ 90 Plate:2
- Mate:211: 4040 1ft:2 ↔ 90 Plate:4
- Flush:104 (2 mm): 4080 6ft:1 ↔ 4 Hole Bracket:40
- Flush:105 (2 mm): 4080 6ft:1 ↔ 4 Hole Bracket:39
- Flush:106 (2 mm): 4080 6ft:2 ↔ 4 Hole Bracket:30
- Flush:107 (2 mm): 4080 6ft:2 ↔ 4 Hole Bracket:29
- Flush:108 (2 mm): 4080 6ft:1 ↔ 4 Hole Bracket:42
- Flush:109 (2 mm): 4080 6ft:1 ↔ 4 Hole Bracket:41
- Flush:110 (2 mm): 4080 6ft:2 ↔ 4 Hole Bracket:28
- Flush:111 (2 mm): 4080 6ft:2 ↔ 4 Hole Bracket:27
- Mate:212: 4080 6ft:1 ↔ 4080 2.5ft:1
- Flush:112: 4080 6ft:1 ↔ 4080 2.5ft:1
- Mate:213: 4 Hole Bracket:40 ↔ 4080 2.5ft:1
- Mate:214: 4 Hole Bracket:39 ↔ 4080 2.5ft:1
- Mate:215: 4 Hole Bracket:29 ↔ 4080 2.5ft:1
- Mate:216: 4 Hole Bracket:30 ↔ 4080 2.5ft:1
- Mate:217: 4080 6ft:1 ↔ 8080 2.5ft:3
- Flush:113: 4080 6ft:1 ↔ 8080 2.5ft:3
- Mate:218: 4 Hole Bracket:42 ↔ 8080 2.5ft:3
- Mate:219: 4 Hole Bracket:41 ↔ 8080 2.5ft:3
- Mate:220: 4 Hole Bracket:27 ↔ 8080 2.5ft:3
- Mate:221: 4 Hole Bracket:28 ↔ 8080 2.5ft:3
- Mate:226: 4040 angled:1 ↔ 8080 2.5ft:3
- Mate:227: 4040 1ft:2 ↔ 4080 2.5ft:1
- Flush:116: 4040 1ft:2 ↔ 4080 2.5ft:1
- Mate:228: 4040 1ft:2 ↔ 90 Plate:4
- Mate:229: 4040 1ft:1 ↔ 90 Plate:2
- Mate:230: 90 Plate:2 ↔ 4080 2.5ft:1
- Mate:231: 90 Plate:4 ↔ 4080 2.5ft:1
- Flush:117: 4040 1.5ft:1 ↔ 4080 2.5ft:1
- Flush:118: 4040 1.5ft:1 ↔ ODSY-0007-001:1
- Flush:119: 4040 1ft:2 ↔ ODSY-0007-001:1
- Mate:232: 4040 1ft:2 ↔ ODSY-0007-001:1
- Mate:233: ODSY-0007-003:1 ↔ 8080 2.5ft:1
- Mate:241: 4080 6ft:1 ↔ 4040 2.5ft:8
- Mate:242: 4080 6ft:1 ↔ 4040 2.5ft:9
- Flush:122: 4080 6ft:1 ↔ 4040 2.5ft:9
- Flush:123: 4080 6ft:1 ↔ 4040 2.5ft:8
- Mate:244: 4040 2.5ft:8 ↔ 4 Hole Bracket:45
- Flush:124 (2 mm): 4040 2.5ft:8 ↔ 4 Hole Bracket:45
- Mate:245: 4080 6ft:2 ↔ 4 Hole Bracket:45
- Mate:246: 4040 2.5ft:8 ↔ 4 Hole Bracket:46
- Flush:125 (2 mm): 4040 2.5ft:8 ↔ 4 Hole Bracket:46
- Mate:247: 4080 6ft:2 ↔ 4 Hole Bracket:46
- Mate:248: 4040 2.5ft:9 ↔ 4 Hole Bracket:48
- Flush:126 (2 mm): 4040 2.5ft:9 ↔ 4 Hole Bracket:48
- Mate:249: 4080 6ft:2 ↔ 4 Hole Bracket:48
- Mate:250: 4040 2.5ft:9 ↔ 4 Hole Bracket:49
- Flush:127 (2 mm): 4040 2.5ft:9 ↔ 4 Hole Bracket:49
- Mate:251: 4080 6ft:2 ↔ 4 Hole Bracket:49
- Mate:256: 4040 2.5ft:8 ↔ 4 Hole Bracket:52
- Flush:130 (2 mm): 4040 2.5ft:8 ↔ 4 Hole Bracket:52
- Mate:257: 4080 6ft:1 ↔ 4 Hole Bracket:52
- Mate:258: 4040 2.5ft:8 ↔ 4 Hole Bracket:51
- Flush:131 (2 mm): 4040 2.5ft:8 ↔ 4 Hole Bracket:51
- Mate:259: 4080 6ft:1 ↔ 4 Hole Bracket:51
- Mate:260: 4040 2.5ft:9 ↔ 4 Hole Bracket:56
- Flush:132 (2 mm): 4040 2.5ft:9 ↔ 4 Hole Bracket:56
- Mate:261: 4080 6ft:1 ↔ 4 Hole Bracket:56
- Mate:262: 4040 2.5ft:9 ↔ 4 Hole Bracket:55
- Flush:133 (-2 mm): 4040 2.5ft:9 ↔ 4 Hole Bracket:55
- Mate:263: 4080 6ft:1 ↔ 4 Hole Bracket:55
- Mate:268: ODSY-0007-002:1 ↔ Combustion Chamber Assembly:1
- Mate:269: ODSY-0007-002:1 ↔ Combustion Chamber Assembly:1
- Mate:275: ODSY-0007-001:1 ↔ Load Cell:1
- Mate:276: ODSY-0007-001:1 ↔ Load Cell:1
- Mate:279: ODSY-0007-003:2 ↔ Odyssey Bushing:2
- Mate:280: ODSY-0007-003:2 ↔ Odyssey Bushing:2
- Mate:281: ODSY-0007-003:2 ↔ Odyssey Bushing:2
- Mate:282: ODSY-0007-003:1 ↔ Odyssey Bushing:4
- Mate:283: ODSY-0007-003:1 ↔ Odyssey Bushing:4
- Mate:284: ODSY-0007-003:1 ↔ Odyssey Bushing:4
- Mate:285: ODSY-0007-003:1 ↔ Odyssey Bushing:3
- Mate:286: ODSY-0007-003:1 ↔ Odyssey Bushing:3
- Mate:287: ODSY-0007-003:1 ↔ Odyssey Bushing:3
- Mate:288: ODSY-0007-003:1 ↔ 8080 2.5ft:1
- Mate:289: 4040 2.5ft:5 ↔ ODSY-0007-003:2
- Angle:1 (0 deg): ODSY-0007-003:1 ↔ ODSY-0007-004:1
- Mate:291: ODSY-0007-003:2 ↔ ODSY-0007-004:2
- Mate:292: ODSY-0007-003:2 ↔ ODSY-0007-004:2
- Mate:293: ODSY-0007-003:1 ↔ ODSY-0007-004:1
- Mate:294: ODSY-0007-003:1 ↔ ODSY-0007-004:1
- Mate:295: ODSY-0007-004:1 ↔ Odyssey Bushing:6
- Mate:296: ODSY-0007-004:1 ↔ Odyssey Bushing:6
- Mate:297: ODSY-0007-004:1 ↔ Odyssey Bushing:6
- Mate:298: ODSY-0007-004:1 ↔ Odyssey Bushing:5
- Mate:299: ODSY-0007-004:1 ↔ Odyssey Bushing:5
- Mate:300: ODSY-0007-004:1 ↔ Odyssey Bushing:5
- Mate:301: ODSY-0007-004:2 ↔ Odyssey Bushing:8
- Mate:302: ODSY-0007-004:2 ↔ Odyssey Bushing:8
- Mate:303: ODSY-0007-004:2 ↔ Odyssey Bushing:8
- Mate:304: ODSY-0007-004:2 ↔ Odyssey Bushing:7
- Mate:305: ODSY-0007-004:2 ↔ Odyssey Bushing:7
- Mate:306: ODSY-0007-004:2 ↔ Odyssey Bushing:7
- Mate:307: ODSY-0007-003:1 ↔ 95412A566 Short Threaded Rod:2
- Mate:308: ODSY-0007-003:1 ↔ 95412A566 Short Threaded Rod:4
- Mate:309: ODSY-0007-003:2 ↔ 95412A566 Short Threaded Rod:3
- Mate:310: ODSY-0007-003:2 ↔ 95412A566 Short Threaded Rod:1
- Mate:311: ODSY-0007-003:2 ↔ 95412A566 Short Threaded Rod:1
- Mate:312: ODSY-0007-003:1 ↔ 95412A566 Short Threaded Rod:2
- Mate:313: ODSY-0007-003:1 ↔ 95412A566 Short Threaded Rod:4
- Mate:314: ODSY-0007-003:2 ↔ 95412A566 Short Threaded Rod:3
- Mate:319: ODSY-0007-004:2 ↔ 98804A029 Long Threaded Rod:1
- Mate:320: ODSY-0007-004:2 ↔ 98804A029 Long Threaded Rod:2
- Mate:331: ODSY-0007-001:1 ↔ 92196A801 Load Cell Bolt:1
- Mate:332: ODSY-0007-001:1 ↔ 92196A801 Load Cell Bolt:2
- Mate:333: 92196A801 Load Cell Bolt:1 ↔ 92141A029 0.25 Washer:1
- Mate:334: ODSY-0007-001:1 ↔ 92141A029 0.25 Washer:1
- Mate:335: 92196A801 Load Cell Bolt:1 ↔ 92141A029 0.25 Washer:1
- Mate:336: 92196A801 Load Cell Bolt:2 ↔ 92141A029 0.25 Washer:2
- Mate:337: ODSY-0007-001:1 ↔ 92141A029 0.25 Washer:2
- Mate:338: 92196A801 Load Cell Bolt:2 ↔ 92141A029 0.25 Washer:2
- Mate:339: 92196A801 Load Cell Bolt:2 ↔ 92141A029 0.25 Washer:4
- Mate:341: 92196A801 Load Cell Bolt:1 ↔ 92141A029 0.25 Washer:3
- Mate:342: ODSY-0007-002:1 ↔ 92141A029 0.25 Washer:3
- Mate:343: 4040 angled:1 ↔ 8080 2.5ft:3
- Mate:344: 95412A566 Short Threaded Rod:1 ↔ 92141A029 0.25 Washer:7
- Mate:345: ODSY-0007-004:2 ↔ 92141A029 0.25 Washer:7
- Mate:346: 95412A566 Short Threaded Rod:3 ↔ 92141A029 0.25 Washer:5
- Mate:347: ODSY-0007-004:2 ↔ 92141A029 0.25 Washer:5
- Mate:348: 95412A566 Short Threaded Rod:2 ↔ 92141A029 0.25 Washer:6
- Mate:349: 95412A566 Short Threaded Rod:4 ↔ 92141A029 0.25 Washer:8
- Mate:350: ODSY-0007-004:1 ↔ 92141A029 0.25 Washer:8
- Mate:351: ODSY-0007-004:1 ↔ 92141A029 0.25 Washer:6